# Autodesk Inventor assembly: ASM Frame
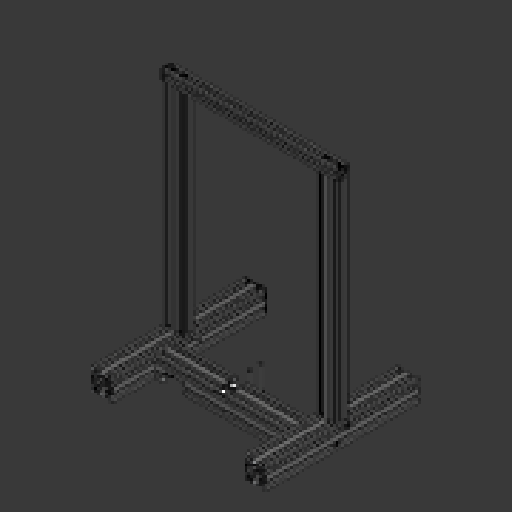
[picture p0: Inventor's stored thumbnail of the model, 512x512]
Saved by Autodesk Inventor 2023 (Build 270158000, 158)
## iProperties
Created: 2018-08-16
Part Number: ASM Frame
Document SubType Name: Assembly
Designer: alber
Sending System: SolidWorks 2015
Last Author: Poseidon
Last Saved: 2018-08-17
Author: alber
## Documents named in this file (8)
- C:\Users\alber\Desktop\Files\Ender3-Upgrade\CAD\ASM Frame.iam
- C:\Users\alber\Desktop\Files\Ender3-Upgrade\CAD\4040 profile.ipt
- C:\Users\alber\Desktop\Files\Ender3-Upgrade\CAD\4040-3 profile.ipt
- C:\Users\alber\Desktop\Files\Ender3-Upgrade\CAD\2020-2 profile.ipt
- C:\Users\alber\Desktop\Files\Ender3-Upgrade\CAD\2040-3R profile.ipt
- C:\Users\alber\Desktop\Files\Ender3-Upgrade\CAD\2040-3L profile.ipt
- C:\Users\alber\Desktop\Files\Ender3-Upgrade\CAD\2020 Endcap.ipt
- C:\Users\alber\Desktop\Files\Ender3-Upgrade\CAD\M5X45 Socket Head Screw.ipt
## Components (25 placed, 7 different names)
1. 4040 profile:1 — Mate:1, Flush:1, Flush:5, Insert:1
2. 4040 profile:2 — Mate:3, Flush:4, Flush:5
3. 4040-3 profile:1 — Mate:1, Flush:1, Insert:1
4. 2020-2 profile:1 — Flush:2, Mate:2, Flush:3
5. 2040-3R profile:1
6. 2040-3L profile:1 — Flush:2, Mate:2, Flush:3, Mate:3, Flush:4
7. 2020 Endcap:1
8. 2020 Endcap:2
9. 2020 Endcap:4
10. M5X45 Socket Head Screw:1
11. M5X45 Socket Head Screw:2
12. M5X45 Socket Head Screw:3
13. M5X45 Socket Head Screw:4
14. M5X45 Socket Head Screw:5
15. M5X45 Socket Head Screw:6
16. M5X45 Socket Head Screw:7
17. M5X45 Socket Head Screw:8
18. M5X45 Socket Head Screw:9
19. M5X45 Socket Head Screw:10
20. M5X45 Socket Head Screw:12
21. M5X45 Socket Head Screw:13
22. M5X45 Socket Head Screw:14
23. 2020 Endcap:5
24. 2020 Endcap:6
25. 2020 Endcap:7
## Relationships (9: Flush 5, Mate 3, Insert 1)
- Mate:1: 4040 profile:1 ↔ 4040-3 profile:1
- Flush:1: 4040 profile:1 ↔ 4040-3 profile:1
- Flush:2: 2020-2 profile:1 ↔ 2040-3L profile:1
- Mate:2: 2020-2 profile:1 ↔ 2040-3L profile:1
- Flush:3: 2020-2 profile:1 ↔ 2040-3L profile:1
- Mate:3: 4040 profile:2 ↔ 2040-3L profile:1
- Flush:4: 4040 profile:2 ↔ 2040-3L profile:1
- Flush:5: 4040 profile:1 ↔ 4040 profile:2
- Insert:1: 4040 profile:1 ↔ 4040-3 profile:1
